# Autodesk Inventor assembly: AssyClimber
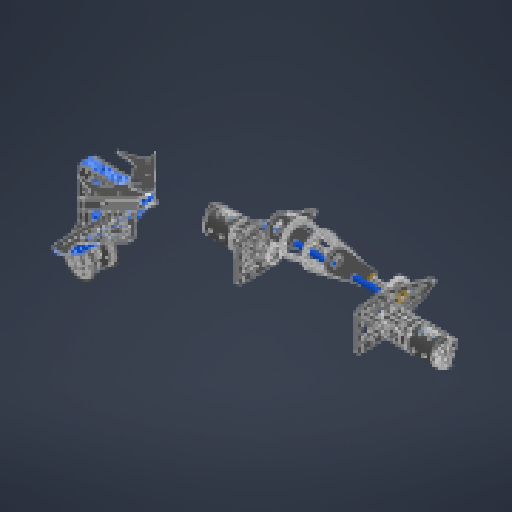
[picture p0: Inventor's stored thumbnail of the model, 512x512]
Saved by Autodesk Inventor 2024.3 (Build 283343000, 343)
## iProperties
Created: 2025-03-19
Part Number: AssyClimber
Document SubType Name: Assembly
Designer: jings
Author: jings
## Documents named in this file (7)
- C:\Users\jings\OneDrive\Desktop\FRC 5885\2025-Poseidon-Mechanical\climber\AssyClimber.iam
- C:\Users\jings\Downloads\CageNoChain\ClimberBottomBrace\ClimberBottomBrace.ipt
- C:\Users\jings\Downloads\CageNoChain\ClimberFrame\ClimberFrame.ipt
- C:\Users\jings\Downloads\CageNoChain\ClimberHook1\ClimberHook1.ipt
- C:\Users\jings\Downloads\CageNoChain\ClimberHook2\ClimberHook2.ipt
- C:\Users\jings\Downloads\ClimberDriving\ClimberDriving\ClimberDriving.ipt
- C:\Users\jings\OneDrive\Desktop\FRC 5885\2025-Poseidon-Mechanical\climber\ClimberAxel.ipt
## Components (6 placed, 6 different names)
1. ClimberDriving:1 — Insert:6
2. ClimberAxel:1
3. ClimberBottomBrace:1 — Insert:3, Insert:4
4. ClimberFrame:1 — Insert:1, Insert:2, Insert:3, Insert:4, Insert:6
5. ClimberHook1:1 — Insert:1
6. ClimberHook2:1 — Insert:2
## Relationships (5: Insert 5)
- Insert:1: ClimberFrame:1 ↔ ClimberHook1:1
- Insert:2: ClimberFrame:1 ↔ ClimberHook2:1
- Insert:3: ClimberBottomBrace:1 ↔ ClimberFrame:1
- Insert:4: ClimberBottomBrace:1 ↔ ClimberFrame:1
- Insert:6: ClimberDriving:1 ↔ ClimberFrame:1
